# Autodesk Inventor assembly: am-4668 2 Stage Climber in a Box2
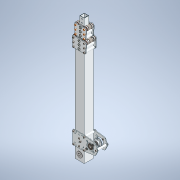
[picture p0: Inventor's stored thumbnail of the model, 180x180]
Saved by Autodesk Inventor 2022 (Build 260153000, 153)
## iProperties
Created: 2022-02-03
Part Number: am-4668 2 Stage Climber in a Box2
Description: STEP AP214
Document SubType Name: Assembly
Designer: tagaz
Sending System: SolidWorks 2021
Preprocessor: SwSTEP 2.0
Title: am-4668 2 Stage Climber in a Box.STEP
Revision Number: ANY
## Documents named in this file (10)
- C:\Users\tagaz\OneDrive\Documents\T3-Cad\CAD\2022 Parts\TelescopeElev\am-4668 2 Stage Climber in a Box2.iam
- C:\Users\tagaz\Downloads\2x2 Example Tube.ipt
- C:\Users\tagaz\Downloads\1.5x1.5 Example Tube.ipt
- C:\Users\tagaz\Downloads\1x1 Simple Example Tube.ipt
- C:\Users\tagaz\Downloads\am-4664 2IN Winch Kit.iam
- C:\Users\tagaz\Downloads\am-4662 2.0in to 1.5in Climber in a Box Bearing Assembly.iam
- C:\Users\tagaz\Downloads\am-4661 1.5in to 1.0in Tubing Bearing Kit.iam
- C:\Users\tagaz\Downloads\am-4662 1.5in Nylon Bearing Clamp Sub Assembly.iam
- C:\Users\tagaz\Downloads\am-4661 1.0 Nylon Bearing Clamp Sub Assembly.iam
- C:\Users\tagaz\OneDrive\Documents\T3-Cad\CAD\Bearing  for THUNDER.ipt
## Components (10 placed, 9 different names)
1. 2x2 Example Tube_1 — Flush:1, Mate:1, Mate:2, Tangent:1, Mate:8, Mate:9, Insert:1, Insert:2
2. 1.5x1.5 Example Tube_2 — Mate:4, Mate:5, Flush:2, Mate:7, Tangent:2, Mate:12, Mate:13, Mate:14
3. 1x1 Simple Example Tube_3 — Mate:10, Mate:11, Flush:3
4. am-4664 2IN Winch Kit_4 [sub-assembly] — Flush:1
5. am-4662 2.0in to 1.5in Climber in a Box Bearing Assembly_5 [sub-assembly] — Mate:1, Mate:2, Tangent:1
6. am-4661 1.5in to 1.0in Tubing Bearing Kit_6 [sub-assembly] — Mate:4, Mate:7, Tangent:2
7. am-4662 1.5in Nylon Bearing Clamp Sub Assembly_8 [sub-assembly] — Mate:5, Flush:2, Mate:8, Mate:9, Mate:14
8. am-4661 1.0 Nylon Bearing Clamp Sub Assembly_9 [sub-assembly] — Mate:10, Mate:11, Mate:12, Mate:13, Flush:3
9. Bearing  for THUNDER:1 — Insert:2
10. Bearing  for THUNDER:2 — Insert:1
## Relationships (19: Mate 12, Flush 3, Tangent 2, Insert 2)
- Flush:1 (-63.5 mm): 2x2 Example Tube_1 ↔ am-4664 2IN Winch Kit_4
- Mate:1: 2x2 Example Tube_1 ↔ am-4662 2.0in to 1.5in Climber in a Box Bearing Assembly_5
- Mate:2: 2x2 Example Tube_1 ↔ am-4662 2.0in to 1.5in Climber in a Box Bearing Assembly_5
- Tangent:1: 2x2 Example Tube_1 ↔ am-4662 2.0in to 1.5in Climber in a Box Bearing Assembly_5
- Mate:4: 1.5x1.5 Example Tube_2 ↔ am-4661 1.5in to 1.0in Tubing Bearing Kit_6
- Mate:5: 1.5x1.5 Example Tube_2 ↔ am-4662 1.5in Nylon Bearing Clamp Sub Assembly_8
- Flush:2: 1.5x1.5 Example Tube_2 ↔ am-4662 1.5in Nylon Bearing Clamp Sub Assembly_8
- Mate:7: 1.5x1.5 Example Tube_2 ↔ am-4661 1.5in to 1.0in Tubing Bearing Kit_6
- Mate:8 (0.4445 mm): 2x2 Example Tube_1 ↔ am-4662 1.5in Nylon Bearing Clamp Sub Assembly_8
- Mate:9 (0.4445 mm): 2x2 Example Tube_1 ↔ am-4662 1.5in Nylon Bearing Clamp Sub Assembly_8
- Tangent:2: 1.5x1.5 Example Tube_2 ↔ am-4661 1.5in to 1.0in Tubing Bearing Kit_6
- Mate:10: 1x1 Simple Example Tube_3 ↔ am-4661 1.0 Nylon Bearing Clamp Sub Assembly_9
- Mate:11: 1x1 Simple Example Tube_3 ↔ am-4661 1.0 Nylon Bearing Clamp Sub Assembly_9
- Mate:12 (0.4445 mm): 1.5x1.5 Example Tube_2 ↔ am-4661 1.0 Nylon Bearing Clamp Sub Assembly_9
- Mate:13 (0.4445 mm): 1.5x1.5 Example Tube_2 ↔ am-4661 1.0 Nylon Bearing Clamp Sub Assembly_9
- Flush:3: 1x1 Simple Example Tube_3 ↔ am-4661 1.0 Nylon Bearing Clamp Sub Assembly_9
- Mate:14: 1.5x1.5 Example Tube_2 ↔ am-4662 1.5in Nylon Bearing Clamp Sub Assembly_8
- Insert:1: 2x2 Example Tube_1 ↔ Bearing  for THUNDER:2
- Insert:2: 2x2 Example Tube_1 ↔ Bearing  for THUNDER:1
